# Autodesk Inventor assembly: Lidarsee
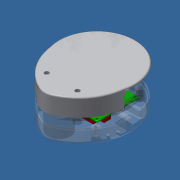
[picture p0: Inventor's stored thumbnail of the model, 180x180]
Saved by Autodesk Inventor 2016 (Build 200138000, 138)
## iProperties
Created: 2017-05-09
Part Number: Lidarsee
Material: Generisch
Document SubType Name: Assembly
Designer: 4ndreas
Author: 4ndreas
## Documents named in this file (6)
- C:\Users\4ndreas\Documents\Inventor\lidarsee\Lidarsee.iam
- C:\Users\4ndreas\Documents\Inventor\lidarsee\LidarseeCase_A.ipt
- C:\Users\4ndreas\Documents\Inventor\lidarsee\Lidar.ipt
- C:\Users\4ndreas\Documents\Inventor\lidarsee\Motherboard_STM32F405RG_simpel.ipt
- C:\Users\4ndreas\Documents\Inventor\lidarsee\LidarseeCase_B.ipt
- C:\Users\4ndreas\Documents\Inventor\lidarsee\LidarseeCase_C.ipt
## Components (5 placed, 5 different names)
1. LidarseeCase_A:1 — Fluchtend:1, Fluchtend:2, Fluchtend:3, Passend:1, Passend:2, Passend:3, Passend:4, Passend:7, Passend:8, Passend:9, Passend:10, Passend:13, Passend:14
2. Lidar:1 — Passend:1, Passend:2, Passend:3, Passend:11, Passend:12
3. Motherboard_STM32F405RG_simpel:1 — Passend:4, Passend:13, Passend:14
4. LidarseeCase_B:1 — Passend:7, Passend:8, Passend:9
5. LidarseeCase_C:1 — Passend:10, Passend:11, Passend:12
## Relationships (15: Mate 12, Flush 3)
- Fluchtend:1 [Flush]: LidarseeCase_A:1
- Fluchtend:2 [Flush]: LidarseeCase_A:1
- Fluchtend:3 [Flush]: LidarseeCase_A:1
- Passend:1 [Mate]: LidarseeCase_A:1 ↔ Lidar:1
- Passend:2 [Mate]: LidarseeCase_A:1 ↔ Lidar:1
- Passend:3 [Mate]: LidarseeCase_A:1 ↔ Lidar:1
- Passend:4 [Mate] (2 mm): LidarseeCase_A:1 ↔ Motherboard_STM32F405RG_simpel:1
- Passend:7 [Mate]: LidarseeCase_A:1 ↔ LidarseeCase_B:1
- Passend:8 [Mate]: LidarseeCase_A:1 ↔ LidarseeCase_B:1
- Passend:9 [Mate]: LidarseeCase_A:1 ↔ LidarseeCase_B:1
- Passend:10 [Mate]: LidarseeCase_A:1 ↔ LidarseeCase_C:1
- Passend:11 [Mate]: Lidar:1 ↔ LidarseeCase_C:1
- Passend:12 [Mate]: Lidar:1 ↔ LidarseeCase_C:1
- Passend:13 [Mate]: LidarseeCase_A:1 ↔ Motherboard_STM32F405RG_simpel:1
- Passend:14 [Mate]: LidarseeCase_A:1 ↔ Motherboard_STM32F405RG_simpel:1
